# Autodesk Inventor assembly: AKK RS2205 2300KV
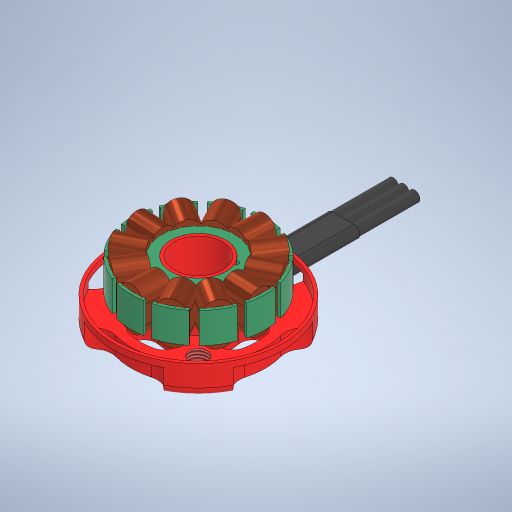
[picture p0: Inventor's stored thumbnail of the model, 512x512]
Saved by Autodesk Inventor 2023.2 (Build 272271000, 271)
## iProperties
Created: 2024-01-31
Part Number: AKK RS2205 2300KV
Document SubType Name: Assembly
Designer: Nathan Cai
Author: Nathan Cai
## Documents named in this file (11)
- E:\Documents\Inventor\Blipper V1\AKK RS2205 2300KV\AKK RS2205 2300KV.iam
- E:\Documents\Inventor\Blipper V1\AKK RS2205 2300KV\BASE.ipt
- E:\Documents\Inventor\Blipper V1\AKK RS2205 2300KV\BEARING.ipt
- E:\Documents\Inventor\Blipper V1\AKK RS2205 2300KV\STATOR.ipt
- E:\Documents\Inventor\Blipper V1\AKK RS2205 2300KV\COILS.ipt
- E:\Documents\Inventor\Blipper V1\AKK RS2205 2300KV\CAN.ipt
- E:\Documents\Inventor\Blipper V1\AKK RS2205 2300KV\98541A111_External Retaining Ring\98541A111_External Retaining Ring.ipt
- E:\Documents\Inventor\Blipper V1\AKK RS2205 2300KV\Magnets.ipt
- E:\Documents\Inventor\Blipper V1\AKK RS2205 2300KV\Cable Sleeve.ipt
- E:\Documents\Inventor\Blipper V1\AKK RS2205 2300KV\SHAFT.ipt
- E:\Documents\Inventor\Blipper V1\AKK RS2205 2300KV\SPACER.ipt
## Components (35 placed, 10 different names)
1. 98541A111_External Retaining Ring:1 — Mate:17
2. SPACER:1 — Mate:16, Mate:17
3. SHAFT:1
4. BASE:1 — Mate:1, Flush:1, Mate:2, Flush:2, Mate:3, Flush:3, Mate:15, Tangent:5, Flush:4
5. BEARING:1 — Mate:1, Flush:1, Mate:7, Mate:16
6. BEARING:2 — Mate:2, Flush:2, Mate:6
7. STATOR:1 — Mate:3, Flush:3, Tangent:1, Mate:4, Mate:5, Tangent:2
8. CAN:1 — Mate:6, Mate:7, Mate:14, Tangent:3, Tangent:4
9. Cable Sleeve:1 — Mate:15, Tangent:5, Flush:4
10. COILS:1 — Tangent:1, Mate:4, Mate:5, Tangent:2
11. COILS:2
12. COILS:3
13. COILS:4
14. COILS:5
15. COILS:6
16. COILS:7
17. COILS:8
18. COILS:9
19. COILS:10
20. COILS:11
21. COILS:12
22. Magnets:1 — Mate:14, Tangent:3, Tangent:4
23. Magnets:2
24. Magnets:3
25. Magnets:4
26. Magnets:5
27. Magnets:6
28. Magnets:7
29. Magnets:8
30. Magnets:9
31. Magnets:10
32. Magnets:11
33. Magnets:12
34. Magnets:13
35. Magnets:14
## Component patterns: (12 elements, first: COILS:1), (14 elements, first: Magnets:1)
## Relationships (24: Mate 15, Tangent 5, Flush 4)
- Mate:1: BASE:1 ↔ BEARING:1
- Flush:1: BASE:1 ↔ BEARING:1
- Mate:2: BASE:1 ↔ BEARING:2
- Flush:2: BASE:1 ↔ BEARING:2
- Mate:3: BASE:1 ↔ STATOR:1
- Flush:3: BASE:1 ↔ STATOR:1
- Tangent:1: STATOR:1 ↔ COILS:1
- Mate:4: STATOR:1 ↔ COILS:1
- Mate:5: STATOR:1 ↔ COILS:1
- Tangent:2: STATOR:1 ↔ COILS:1
- Mate:6: BEARING:2 ↔ CAN:1
- Mate:7: BEARING:1 ↔ CAN:1
- [Mate]: SHAFT:1 ↔ CAN:1
- [Mate]: SHAFT:1 ↔ BEARING:1
- [Mate]: SPACER:1 ↔ SHAFT:1
- [Mate]: 98541A111_External Retaining Ring:1 ↔ SHAFT:1
- Mate:14: CAN:1 ↔ Magnets:1
- Tangent:3: CAN:1 ↔ Magnets:1
- Tangent:4: CAN:1 ↔ Magnets:1
- Mate:15: BASE:1 ↔ Cable Sleeve:1
- Tangent:5: BASE:1 ↔ Cable Sleeve:1
- Flush:4: BASE:1 ↔ Cable Sleeve:1
- Mate:16: SPACER:1 ↔ BEARING:1
- Mate:17: 98541A111_External Retaining Ring:1 ↔ SPACER:1
